# Autodesk Inventor assembly: Rail truck area subassembly
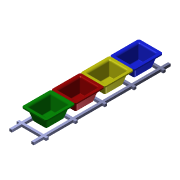
[picture p0: Inventor's stored thumbnail of the model, 180x180]
Saved by Autodesk Inventor 2015 (Build 190159000, 159)
## iProperties
Created: 2015-04-10
Part Number: Rail truck area subassembly
Document SubType Name: Assembly
Designer: Vukica
Author: Vukica
## Documents named in this file (6)
- C:\Users\Vukica\Dropbox\IEEE\hardware rules\2016Hardware_Court_v6\Rail truck area subassembly.iam
- C:\Users\Vukica\Dropbox\IEEE\hardware rules\2016Hardware_Court_v6\Rail zone.ipt
- C:\Users\Vukica\Dropbox\IEEE\hardware rules\2016Hardware_Court_v6\Rail car blue.ipt
- C:\Users\Vukica\Dropbox\IEEE\hardware rules\2016Hardware_Court_v6\Rail car yellow.ipt
- C:\Users\Vukica\Dropbox\IEEE\hardware rules\2016Hardware_Court_v6\Rail car red.ipt
- C:\Users\Vukica\Dropbox\IEEE\hardware rules\2016Hardware_Court_v6\Rail car green.ipt
## Components (5 placed, 5 different names)
1. Rail zone:1 — Mate:1, Mate:2, Mate:4, Mate:6, Flush:4, Flush:5
2. Rail car blue:1 — Mate:1, Mate:3, Flush:1
3. Rail car yellow:1 — Mate:2, Mate:3, Flush:1, Mate:5, Flush:2
4. Rail car red:1 — Mate:4, Mate:5, Flush:2, Mate:7, Flush:3
5. Rail car green:1 — Mate:6, Mate:7, Flush:3, Flush:4, Flush:5
## Relationships (12: Mate 7, Flush 5)
- Mate:1: Rail zone:1 ↔ Rail car blue:1
- Mate:2: Rail zone:1 ↔ Rail car yellow:1
- Mate:3: Rail car blue:1 ↔ Rail car yellow:1
- Flush:1: Rail car blue:1 ↔ Rail car yellow:1
- Mate:4: Rail zone:1 ↔ Rail car red:1
- Mate:5: Rail car yellow:1 ↔ Rail car red:1
- Flush:2: Rail car yellow:1 ↔ Rail car red:1
- Mate:6: Rail zone:1 ↔ Rail car green:1
- Mate:7: Rail car red:1 ↔ Rail car green:1
- Flush:3: Rail car red:1 ↔ Rail car green:1
- Flush:4 (25.4 mm): Rail zone:1 ↔ Rail car green:1
- Flush:5: Rail zone:1 ↔ Rail car green:1
